# Autodesk Inventor assembly: 60SC40D-BG
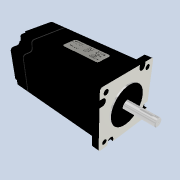
[picture p0: Inventor's stored thumbnail of the model, 180x180]
Saved by Autodesk Inventor 2020 (Build 240168000, 168)
## iProperties
Created: 2020-01-20
Part Number: 60SC40D-BG
Document SubType Name: Assembly
Designer: TES
Author: TES
## Documents named in this file (4)
- E:\PROJEKTE TES\60SC40D-BG.iam
- E:\PROJEKTE TES\60SC40D.ipt
- C:\Users\TES\Documents\Inventor\Content Center Files\R2020\en-US\BS EN ISO 7045 H\EN ISO 7045 - M2 x 3 - 4.8 - H(1).ipt
- C:\Users\TES\Documents\Inventor\Content Center Files\R2020\en-US\BS EN ISO 7045 H\EN ISO 7045 - M2 x 5 - 4.8 - H(1).ipt
## Components (13 placed, 3 different names)
1. 60SC40D:1 — Insert:1, Insert:2, Insert:3, Insert:4, Insert:5, Insert:6, Insert:7, Insert:8, Insert:9, Insert:10, Insert:11, Insert:12
2. BS EN ISO 7045 H - Metric M2 x 3 - 4.8 - H:1 — Insert:1
3. BS EN ISO 7045 H - Metric M2 x 3 - 4.8 - H:2 — Insert:2
4. BS EN ISO 7045 H - Metric M2 x 3 - 4.8 - H:3 — Insert:3
5. BS EN ISO 7045 H - Metric M2 x 3 - 4.8 - H:4 — Insert:4
6. BS EN ISO 7045 H - Metric M2 x 3 - 4.8 - H:5 — Insert:5
7. BS EN ISO 7045 H - Metric M2 x 3 - 4.8 - H:6 — Insert:6
8. BS EN ISO 7045 H - Metric M2 x 3 - 4.8 - H:7 — Insert:7
9. BS EN ISO 7045 H - Metric M2 x 3 - 4.8 - H:8 — Insert:8
10. BS EN ISO 7045 H - Metric M2 x 5 - 4.8 - H:1 — Insert:9
11. BS EN ISO 7045 H - Metric M2 x 5 - 4.8 - H:2 — Insert:10
12. BS EN ISO 7045 H - Metric M2 x 5 - 4.8 - H:3 — Insert:11
13. BS EN ISO 7045 H - Metric M2 x 5 - 4.8 - H:4 — Insert:12
## Relationships (12: Insert 12)
- Insert:1: 60SC40D:1 ↔ BS EN ISO 7045 H - Metric M2 x 3 - 4.8 - H:1
- Insert:2: 60SC40D:1 ↔ BS EN ISO 7045 H - Metric M2 x 3 - 4.8 - H:2
- Insert:3: 60SC40D:1 ↔ BS EN ISO 7045 H - Metric M2 x 3 - 4.8 - H:3
- Insert:4: 60SC40D:1 ↔ BS EN ISO 7045 H - Metric M2 x 3 - 4.8 - H:4
- Insert:5: 60SC40D:1 ↔ BS EN ISO 7045 H - Metric M2 x 3 - 4.8 - H:5
- Insert:6: 60SC40D:1 ↔ BS EN ISO 7045 H - Metric M2 x 3 - 4.8 - H:6
- Insert:7: 60SC40D:1 ↔ BS EN ISO 7045 H - Metric M2 x 3 - 4.8 - H:7
- Insert:8: 60SC40D:1 ↔ BS EN ISO 7045 H - Metric M2 x 3 - 4.8 - H:8
- Insert:9: 60SC40D:1 ↔ BS EN ISO 7045 H - Metric M2 x 5 - 4.8 - H:1
- Insert:10: 60SC40D:1 ↔ BS EN ISO 7045 H - Metric M2 x 5 - 4.8 - H:2
- Insert:11: 60SC40D:1 ↔ BS EN ISO 7045 H - Metric M2 x 5 - 4.8 - H:3
- Insert:12: 60SC40D:1 ↔ BS EN ISO 7045 H - Metric M2 x 5 - 4.8 - H:4
